# Autodesk Inventor assembly: y-carriage-double
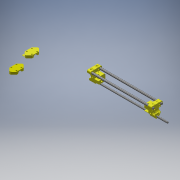
[picture p0: Inventor's stored thumbnail of the model, 180x180]
Saved by Autodesk Inventor 2019.4 (Build 234330000, 330)
## iProperties
Created: 2020-08-29
Part Number: y-carriage-double
Material: Generisch
Document SubType Name: Assembly
Designer: marc
Author: marc
## Documents named in this file (7)
- C:\Users\marc\Google Drive\Projekte\3D Drucker\brezzlicator\1. Printed Parts\3. Modified by marc\y-carriage-double.iam
- C:\Users\marc\Google Drive\Projekte\3D Drucker\brezzlicator\1. Printed Parts\2. Inventor Parts\Linear rail - Y.ipt
- C:\Users\marc\Google Drive\Projekte\3D Drucker\brezzlicator\1. Printed Parts\2. Inventor Parts\Linear rail - X.ipt
- C:\Users\marc\Google Drive\Projekte\3D Drucker\brezzlicator\1. Printed Parts\2. Inventor Parts\Y Carriage Clamp 1.0.ipt
- C:\Users\marc\Google Drive\Projekte\3D Drucker\brezzlicator\1. Printed Parts\3. Modified by marc\Y Carriage 2.0_A.ipt
- C:\Users\marc\Google Drive\Projekte\3D Drucker\brezzlicator\1. Printed Parts\3. Modified by marc\Y Carriage 2.0_B.ipt
- C:\Users\marc\Google Drive\Projekte\3D Drucker\brezzlicator\1. Printed Parts\3. Modified by marc\titan_direct_drive_extruder\y_clamp_with_endstop_flag.ipt
## Components (7 placed, 6 different names)
1. Linear rail - Y:1 — Starr:1
2. Linear rail - Y:2 — Starr:2, Starr:3
3. Linear rail - X:1 — Drehbar:1
4. Y Carriage Clamp 1.0:1
5. Y Carriage 2.0_A:1 — Starr:1, Starr:2, Drehbar:1
6. Y Carriage 2.0_B:1 — Starr:3
7. y_clamp_with_endstop_flag:1
## Relationships (4: WeldJoint 3, RevoluteJoint 1)
- Starr:1 [WeldJoint]: Linear rail - Y:1 ↔ Y Carriage 2.0_A:1
- Starr:2 [WeldJoint]: Linear rail - Y:2 ↔ Y Carriage 2.0_A:1
- Drehbar:1 [RevoluteJoint]: Linear rail - X:1 ↔ Y Carriage 2.0_A:1
- Starr:3 [WeldJoint] (-22.75 mm): Linear rail - Y:2 ↔ Y Carriage 2.0_B:1
